# Autodesk Inventor assembly: hook block
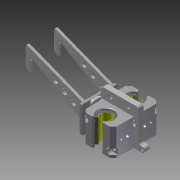
[picture p0: Inventor's stored thumbnail of the model, 180x180]
Saved by Autodesk Inventor 2013 (Build 170138000, 138)
## iProperties
Created: 2013-01-27
Part Number: hook block
Document SubType Name: Assembly
Designer: Arpan
Mass: 1798.72 g
Surface Area: 1895.83 cm^2
Volume: 596.859 cm^3
Density: 3.01364 g/cm^3
Author: Arpan
## Documents named in this file (6)
- C:\Users\Moses\Documents\GitHub\frc2013CAD\Cimber actual\hook block.iam
- C:\Users\Moses\Documents\GitHub\frc2013CAD\Cimber actual\Bearing Block long style.iam
- C:\Users\Moses\Documents\GitHub\frc2013CAD\Cimber actual\hook mount plate 2.ipt
- C:\Users\Moses\Documents\GitHub\frc2013CAD\Cimber actual\hook mount plate.ipt
- C:\Users\Moses\Documents\GitHub\frc2013CAD\Cimber actual\hook faceplate.ipt
- C:\Users\Moses\Documents\GitHub\frc2013CAD\Cimber actual\hook.ipt
## Components (7 placed, 5 different names)
1. Bearing Block long style:1 [sub-assembly] — Flush:1, Mate:3, Mate:4
2. Bearing Block long style:2 [sub-assembly] — Flush:1, Mate:1, Mate:2
3. hook mount plate 2:1 — Mate:3, Mate:4, Mate:5, Flush:2, Flush:3, Flush:5, Mate:6
4. hook mount plate:1 — Mate:1, Mate:2, Mate:5, Flush:2, Flush:3, Flush:4
5. hook faceplate:1 — Mate:6, Flush:4, Flush:5, Mate:7, Mate:8, Mate:9, Mate:10, Mate:11, Mate:12
6. hook:1 — Mate:10, Mate:11, Mate:12
7. hook:2 — Mate:7, Mate:8, Mate:9
## Relationships (17: Mate 12, Flush 5)
- Flush:1: Bearing Block long style:1 ↔ Bearing Block long style:2
- Mate:1: Bearing Block long style:2 ↔ hook mount plate:1
- Mate:2: Bearing Block long style:2 ↔ hook mount plate:1
- Mate:3: Bearing Block long style:1 ↔ hook mount plate 2:1
- Mate:4: Bearing Block long style:1 ↔ hook mount plate 2:1
- Mate:5: hook mount plate 2:1 ↔ hook mount plate:1
- Flush:2: hook mount plate 2:1 ↔ hook mount plate:1
- Flush:3: hook mount plate 2:1 ↔ hook mount plate:1
- Mate:6: hook mount plate 2:1 ↔ hook faceplate:1
- Flush:4 (-38.1 mm): hook mount plate:1 ↔ hook faceplate:1
- Flush:5: hook mount plate 2:1 ↔ hook faceplate:1
- Mate:7: hook faceplate:1 ↔ hook:2
- Mate:8: hook faceplate:1 ↔ hook:2
- Mate:9: hook faceplate:1 ↔ hook:2
- Mate:10: hook faceplate:1 ↔ hook:1
- Mate:11: hook faceplate:1 ↔ hook:1
- Mate:12: hook faceplate:1 ↔ hook:1
